# Autodesk Inventor assembly: Desenho da Montagem
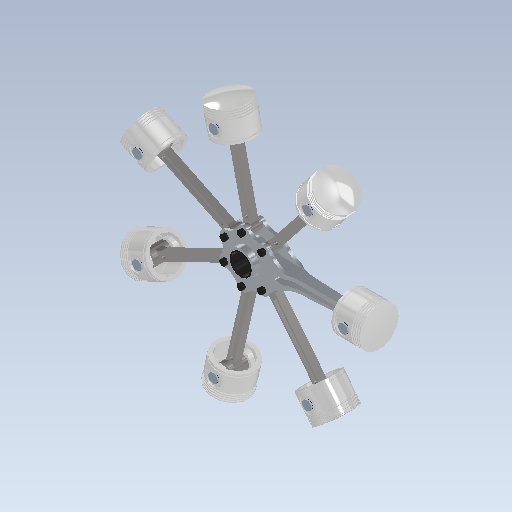
[picture p0: Inventor's stored thumbnail of the model, 512x512]
Saved by Autodesk Inventor 2021 (Build 250183000, 183)
## iProperties
Category: 10
Company: UFABC
Created: 2021-07-24
Document SubType Name: Assembly
Designer: Giovanni
Checked By: Prof. Luis
User Status: 1:7
Description: 2
Author: Giovanni Rodrigues Dias
Title: Desenho da Montagem
Keywords: 2
## Documents named in this file (5)
- C:\Users\irineu\Documents\Inventor\MotorRadial7\MotorPistaoEquipado.iam
- C:\Users\irineu\Documents\Inventor\MotorRadial7\BielaMestraEquipada.iam
- C:\Users\irineu\Documents\Inventor\MotorRadial7\BielaArticuladaEquipada.iam
- C:\Users\irineu\Documents\Inventor\MotorRadial7\PistaoEquipado.iam
- C:\Users\irineu\Documents\Inventor\MotorRadial7\Pino de Ligação.ipt
## Components (20 placed, 4 different names)
1. BielaMestraEquipada:1 [sub-assembly] — Inserir:1, Ângulo:1, Inserir:2, Inserir:3, Inserir:4, Inserir:5, Inserir:6, Coincidente:1, Alinhado:1, Inserir:7, Inserir:8, Inserir:9, Inserir:10, Inserir:11, Inserir:12
2. BielaArticuladaEquipada:1 [sub-assembly] — Inserir:1, Ângulo:1, Ângulo:2, Coincidente:3, Alinhado:3
3. BielaArticuladaEquipada:2 [sub-assembly] — Inserir:3, Ângulo:3, Ângulo:4, Coincidente:7, Alinhado:5
4. BielaArticuladaEquipada:3 [sub-assembly] — Inserir:4, Ângulo:4, Ângulo:5, Coincidente:8, Alinhado:7
5. BielaArticuladaEquipada:4 [sub-assembly] — Inserir:6, Ângulo:6, Coincidente:12, Coincidente:13
6. BielaArticuladaEquipada:5 [sub-assembly] — Inserir:5, Ângulo:5, Ângulo:6, Coincidente:9, Coincidente:10
7. BielaArticuladaEquipada:6 [sub-assembly] — Inserir:2, Ângulo:2, Ângulo:3, Coincidente:4, Coincidente:5
8. PistaoEquipado:1 [sub-assembly] — Coincidente:1, Coincidente:2, Alinhado:2
9. PistaoEquipado:2 [sub-assembly] — Coincidente:3, Alinhado:3, Alinhado:4
10. PistaoEquipado:3 [sub-assembly] — Coincidente:4, Coincidente:5, Coincidente:6
11. PistaoEquipado:4 [sub-assembly] — Coincidente:7, Alinhado:5, Alinhado:6
12. PistaoEquipado:5 [sub-assembly] — Coincidente:8, Alinhado:7, Alinhado:8
13. PistaoEquipado:6 [sub-assembly] — Coincidente:9, Coincidente:10, Coincidente:11
14. PistaoEquipado:7 [sub-assembly] — Coincidente:12, Coincidente:13, Coincidente:14
15. Pino de Ligação:1 — Inserir:7
16. Pino de Ligação:2 — Inserir:8
17. Pino de Ligação:3 — Inserir:9
18. Pino de Ligação:4 — Inserir:10
19. Pino de Ligação:5 — Inserir:11
20. Pino de Ligação:6 — Inserir:12
## Relationships (40: Mate 14, Insert 12, Flush 8, Angle 6)
- Inserir:1: BielaMestraEquipada:1 ↔ BielaArticuladaEquipada:1
- Ângulo:1 [Angle] (51.43 deg): BielaMestraEquipada:1 ↔ BielaArticuladaEquipada:1
- Inserir:2: BielaMestraEquipada:1 ↔ BielaArticuladaEquipada:6
- Ângulo:2 [Angle] (51.43 deg): BielaArticuladaEquipada:1 ↔ BielaArticuladaEquipada:6
- Inserir:3: BielaMestraEquipada:1 ↔ BielaArticuladaEquipada:2
- Ângulo:3 [Angle] (51.43 deg): BielaArticuladaEquipada:2 ↔ BielaArticuladaEquipada:6
- Inserir:4: BielaMestraEquipada:1 ↔ BielaArticuladaEquipada:3
- Ângulo:4 [Angle] (51.43 deg): BielaArticuladaEquipada:2 ↔ BielaArticuladaEquipada:3
- Inserir:5: BielaMestraEquipada:1 ↔ BielaArticuladaEquipada:5
- Ângulo:5 [Angle] (51.43 deg): BielaArticuladaEquipada:3 ↔ BielaArticuladaEquipada:5
- Inserir:6: BielaMestraEquipada:1 ↔ BielaArticuladaEquipada:4
- Ângulo:6 [Angle] (51.43 deg): BielaArticuladaEquipada:4 ↔ BielaArticuladaEquipada:5
- Coincidente:1 [Mate]: BielaMestraEquipada:1 ↔ PistaoEquipado:1
- Alinhado:1 [Flush]: BielaMestraEquipada:1
- Coincidente:2 [Mate]: PistaoEquipado:1
- Alinhado:2 [Flush]: PistaoEquipado:1
- Coincidente:3 [Mate]: BielaArticuladaEquipada:1 ↔ PistaoEquipado:2
- Alinhado:3 [Flush]: BielaArticuladaEquipada:1 ↔ PistaoEquipado:2
- Alinhado:4 [Flush]: PistaoEquipado:2
- Coincidente:4 [Mate]: BielaArticuladaEquipada:6 ↔ PistaoEquipado:3
- Coincidente:5 [Mate]: BielaArticuladaEquipada:6 ↔ PistaoEquipado:3
- Coincidente:6 [Mate]: PistaoEquipado:3
- Coincidente:7 [Mate]: BielaArticuladaEquipada:2 ↔ PistaoEquipado:4
- Alinhado:5 [Flush]: BielaArticuladaEquipada:2 ↔ PistaoEquipado:4
- Alinhado:6 [Flush]: PistaoEquipado:4
- Coincidente:8 [Mate]: BielaArticuladaEquipada:3 ↔ PistaoEquipado:5
- Alinhado:7 [Flush]: BielaArticuladaEquipada:3 ↔ PistaoEquipado:5
- Alinhado:8 [Flush]: PistaoEquipado:5
- Coincidente:9 [Mate]: BielaArticuladaEquipada:5 ↔ PistaoEquipado:6
- Coincidente:10 [Mate]: BielaArticuladaEquipada:5 ↔ PistaoEquipado:6
- Coincidente:11 [Mate]: PistaoEquipado:6
- Coincidente:12 [Mate]: BielaArticuladaEquipada:4 ↔ PistaoEquipado:7
- Coincidente:13 [Mate]: BielaArticuladaEquipada:4 ↔ PistaoEquipado:7
- Coincidente:14 [Mate]: PistaoEquipado:7
- Inserir:7: BielaMestraEquipada:1 ↔ Pino de Ligação:1
- Inserir:8: BielaMestraEquipada:1 ↔ Pino de Ligação:2
- Inserir:9: BielaMestraEquipada:1 ↔ Pino de Ligação:3
- Inserir:10: BielaMestraEquipada:1 ↔ Pino de Ligação:4
- Inserir:11: BielaMestraEquipada:1 ↔ Pino de Ligação:5
- Inserir:12: BielaMestraEquipada:1 ↔ Pino de Ligação:6
